# Autodesk Inventor assembly: SansCapacFata
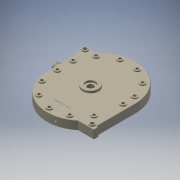
[picture p0: Inventor's stored thumbnail of the model, 180x180]
Saved by Autodesk Inventor 2019 (Build 230136000, 136)
## iProperties
Created: 2019-05-07
Part Number: SansCapacFata
Document SubType Name: Assembly
Designer: forev
Author: forev
## Documents named in this file (4)
- S:\Git_Repositories\Autodesk_Inventor_2019\5. Wankel Engine\SansCapacFata.iam
- S:\Git_Repositories\Autodesk_Inventor_2019\5. Wankel Engine\CapacFata.ipt
- S:\Git_Repositories\Autodesk_Inventor_2019\5. Wankel Engine\Pinion.ipt
- C:\Users\forev\Documents\Inventor\Content Center Files\R2019\en-US\ISO 4762(1)\DIN EN ISO 4762 - M4 x 12.ipt
## Components (8 placed, 3 different names)
1. CapacFata:1 — Mate:1, Mate:2, Angle:1
2. Pinion:1 — Mate:1, Mate:2, Angle:1, Mate:3, Mate:4, Mate:5, Mate:6, Mate:7, Mate:8, Mate:9, Mate:10, Mate:11, Mate:12, Mate:13, Mate:14
3. DIN EN ISO 4762 M4 x 12:1 — Mate:3, Mate:4
4. DIN EN ISO 4762 M4 x 12:2 — Mate:5, Mate:6
5. DIN EN ISO 4762 M4 x 12:3 — Mate:7, Mate:8
6. DIN EN ISO 4762 M4 x 12:4 — Mate:9, Mate:10
7. DIN EN ISO 4762 M4 x 12:5 — Mate:11, Mate:12
8. DIN EN ISO 4762 M4 x 12:6 — Mate:13, Mate:14
## Relationships (15: Mate 14, Angle 1)
- Mate:1: CapacFata:1 ↔ Pinion:1
- Mate:2: CapacFata:1 ↔ Pinion:1
- Angle:1 (99 deg): CapacFata:1 ↔ Pinion:1
- Mate:3: Pinion:1 ↔ DIN EN ISO 4762 M4 x 12:1
- Mate:4: Pinion:1 ↔ DIN EN ISO 4762 M4 x 12:1
- Mate:5: Pinion:1 ↔ DIN EN ISO 4762 M4 x 12:2
- Mate:6: Pinion:1 ↔ DIN EN ISO 4762 M4 x 12:2
- Mate:7: Pinion:1 ↔ DIN EN ISO 4762 M4 x 12:3
- Mate:8: Pinion:1 ↔ DIN EN ISO 4762 M4 x 12:3
- Mate:9: Pinion:1 ↔ DIN EN ISO 4762 M4 x 12:4
- Mate:10: Pinion:1 ↔ DIN EN ISO 4762 M4 x 12:4
- Mate:11: Pinion:1 ↔ DIN EN ISO 4762 M4 x 12:5
- Mate:12: Pinion:1 ↔ DIN EN ISO 4762 M4 x 12:5
- Mate:13: Pinion:1 ↔ DIN EN ISO 4762 M4 x 12:6
- Mate:14: Pinion:1 ↔ DIN EN ISO 4762 M4 x 12:6
